# Autodesk Inventor assembly: pcbwitchElements
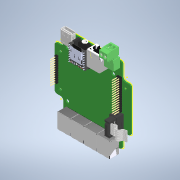
[picture p0: Inventor's stored thumbnail of the model, 180x180]
Saved by Autodesk Inventor 2021 (Build 250183000, 183)
## iProperties
Created: 2023-08-06
Part Number: pcbwitchElements
Document SubType Name: Assembly
Designer: michal
Author: michal
## Documents named in this file (11)
- C:\Users\micha\OneDrive\Dokumenty\GitHub\escape_room_hw_v2\Enclosure\pcbwitchElements.iam
- C:\Users\micha\OneDrive\Dokumenty\GitHub\escape_room_hw_v2\Enclosure\PCB.ipt
- C:\Users\micha\OneDrive\Dokumenty\GitHub\escape_room_hw_v2\Enclosure\Commercial\DFPlayer Mini.iam
- C:\Users\micha\OneDrive\Dokumenty\GitHub\escape_room_hw_v2\Enclosure\Commercial\rjPack.iam
- C:\Users\micha\OneDrive\Dokumenty\GitHub\escape_room_hw_v2\Enclosure\Commercial\power.iam
- C:\Users\micha\OneDrive\Dokumenty\GitHub\escape_room_hw_v2\Enclosure\Commercial\139341875-9-2-338556-1\2-338556-1.ipt
- C:\Users\micha\OneDrive\Dokumenty\GitHub\escape_room_hw_v2\Enclosure\Commercial\J3.iam
- C:\Users\micha\OneDrive\Dokumenty\GitHub\escape_room_hw_v2\Enclosure\Commercial\J9.iam
- C:\Users\micha\OneDrive\Dokumenty\GitHub\escape_room_hw_v2\Enclosure\Commercial\Assembly232.iam
- C:\Users\micha\OneDrive\Dokumenty\GitHub\escape_room_hw_v2\Enclosure\Commercial\Assembly233.iam
- C:\Users\micha\OneDrive\Dokumenty\GitHub\escape_room_hw_v2\Enclosure\Commercial\IDC10Combine2.iam
## Components (10 placed, 10 different names)
1. PCB:1 — Mate:1, Mate:2, Flush:1, Mate:7, Mate:10, Flush:3, Mate:11, Mate:12, Mate:13, Mate:14, Flush:9, Flush:10, Flush:11, Mate:16, Mate:17, Mate:18, Flush:20, Flush:22
2. DFPlayer Mini:1 [sub-assembly] — Mate:7, Flush:10
3. rjPack:1 [sub-assembly] — Mate:10, Flush:3, Flush:22
4. power:1 [sub-assembly] — Mate:11, Flush:6, Flush:9
5. 2-338556-1:1 — Mate:12, Flush:6, Flush:8
6. J3:1 [sub-assembly] — Mate:13, Flush:11
7. J9:1 [sub-assembly] — Mate:14, Flush:8
8. Assembly232:1 [sub-assembly] — Mate:16
9. Assembly233:1 [sub-assembly] — Mate:17, Flush:21
10. IDC10Combine2:1 [sub-assembly] — Mate:18, Flush:20, Flush:21
## Relationships (21: Mate 11, Flush 10)
- Mate:1: PCB:1
- Mate:2: PCB:1
- Flush:1: PCB:1
- Mate:7 (8 mm): PCB:1 ↔ DFPlayer Mini:1
- Mate:10: PCB:1 ↔ rjPack:1
- Flush:3 (-6.4 mm): PCB:1 ↔ rjPack:1
- Mate:11: PCB:1 ↔ power:1
- Mate:12: PCB:1 ↔ 2-338556-1:1
- Flush:6: power:1 ↔ 2-338556-1:1
- Mate:13: PCB:1 ↔ J3:1
- Mate:14: PCB:1 ↔ J9:1
- Flush:8: 2-338556-1:1 ↔ J9:1
- Flush:9 (-4 mm): PCB:1 ↔ power:1
- Flush:10: PCB:1 ↔ DFPlayer Mini:1
- Flush:11: PCB:1 ↔ J3:1
- Mate:16: PCB:1 ↔ Assembly232:1
- Mate:17: PCB:1 ↔ Assembly233:1
- Mate:18: PCB:1 ↔ IDC10Combine2:1
- Flush:20 (9 mm): PCB:1 ↔ IDC10Combine2:1
- Flush:21: Assembly233:1 ↔ IDC10Combine2:1
- Flush:22 (3.6 mm): PCB:1 ↔ rjPack:1
